# Autodesk Inventor assembly: dht22_case
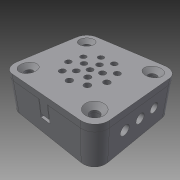
[picture p0: Inventor's stored thumbnail of the model, 180x180]
Saved by Autodesk Inventor 2014 (Build 180170000, 170)
## iProperties
Created: 2016-02-22
Part Number: dht22_case
Document SubType Name: Assembly
Designer: buben
Author: buben
## Documents named in this file (3)
- C:\Users\buben\Documents\dht22-case\case\assemblies\dht22_case.iam
- C:\Users\buben\Documents\dht22-case\case\parts\dht22_case_bottom.ipt
- C:\Users\buben\Documents\dht22-case\case\parts\dht22_case_top.ipt
## Components (2 placed, 2 different names)
1. dht22_case_bottom:1 — Mate:1, Flush:1, Mate:2, Mate:3, Mate:4, Mate:5
2. dht22_case_top:1 — Mate:3, Mate:4, Mate:5
## Relationships (6: Mate 5, Flush 1)
- Mate:1: dht22_case_bottom:1
- Flush:1: dht22_case_bottom:1
- Mate:2: dht22_case_bottom:1
- Mate:3: dht22_case_bottom:1 ↔ dht22_case_top:1
- Mate:4: dht22_case_bottom:1 ↔ dht22_case_top:1
- Mate:5: dht22_case_bottom:1 ↔ dht22_case_top:1
